# Autodesk Inventor assembly: platform_800x500x99_assembly
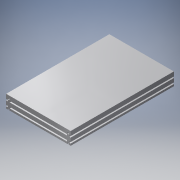
[picture p0: Inventor's stored thumbnail of the model, 180x180]
Saved by Autodesk Inventor 2016 (Build 200138000, 138)
## iProperties
Created: 2015-09-09
Part Number: platform_800x500x99_assembly
Document SubType Name: Assembly
Designer: oscar
Author: oscar
## Documents named in this file (2)
- E:\documents\robocup-at-work\models\arena\elements\platform\service_area\inventor\platform_800x500x99_assembly.iam
- E:\documents\robocup-at-work\models\arena\elements\platform\service_area\inventor\platform_800x500x99.ipt
## Components (1 placed, 1 different names)
1. platform_800x500x99:1 — Mate:1, Flush:1, Mate:2
## Relationships (3: Mate 2, Flush 1)
- Mate:1: platform_800x500x99:1
- Flush:1: platform_800x500x99:1
- Mate:2: platform_800x500x99:1
